# Autodesk Inventor assembly: TimingPulley_S5M_Mechalock
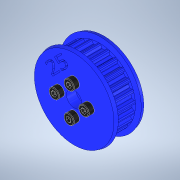
[picture p0: Inventor's stored thumbnail of the model, 180x180]
Saved by Autodesk Inventor 2022 (Build 260153000, 153)
## iProperties
Created: 2022-03-19
Part Number: TimingPulley_S5M_Mechalock
Document SubType Name: Assembly
Designer: satot
Author: satot
## Documents named in this file (6)
- C:\Users\satot\Documents\GrabCAD\NHK2022\BasicParts\TimingPullay\TimingPulley_S5M_Mechalock\TimingPulley_S5M_Mechalock.iam
- C:\Users\satot\Documents\GrabCAD\NHK2022\BasicParts\TimingPullay\TimingPulley_S5M_Mechalock\TimingPulley_S5M_MechaLock_2.ipt
- C:\Users\satot\Documents\GrabCAD\NHK2022\Content Center Files\R2022\ja-JP\六角穴付きボルト\六角穴付きボルト - M3 × 20 - 0.5.ipt
- C:\Users\satot\Documents\GrabCAD\NHK2022\Content Center Files\R2022\ja-JP\スプリング\スプリング - M3 × 0.7.ipt
- C:\Users\satot\Documents\GrabCAD\NHK2022\Content Center Files\R2022\ja-JP\ナット\ナット - M3 × 2.4.ipt
- C:\Users\satot\Documents\GrabCAD\NHK2022\BasicParts\TimingPullay\TimingPulley_S5M_Mechalock\TimingPulley_S5M_MechaLock_1.ipt
## Components (14 placed, 5 different names)
1. TimingPulley_S5M_MechaLock_1:1 — フラッシュ:1, メイト:1, メイト:2, メイト:3, メイト:4, メイト:5, メイト:6, メイト:7, メイト:8, メイト:9, メイト:10, メイト:11, メイト:13, メイト:15, メイト:17
2. TimingPulley_S5M_MechaLock_2:1 — フラッシュ:1, メイト:1, メイト:2, メイト:12, メイト:14, メイト:16, メイト:18
3. 六角穴付きボルト M3 x 20:1 — メイト:3, メイト:4
4. スプリング M3:1 — メイト:11, メイト:12, 挿入:1
5. ナット M3:1 — 挿入:1
6. 六角穴付きボルト M3 x 20:2 — メイト:5, メイト:6
7. 六角穴付きボルト M3 x 20:3 — メイト:7, メイト:8
8. 六角穴付きボルト M3 x 20:4 — メイト:9, メイト:10
9. スプリング M3:2 — メイト:13, メイト:14, 挿入:2
10. スプリング M3:3 — メイト:15, メイト:16, 挿入:3
11. スプリング M3:4 — メイト:17, メイト:18, 挿入:4
12. ナット M3:2 — 挿入:2
13. ナット M3:3 — 挿入:3
14. ナット M3:4 — 挿入:4
## Relationships (23: Mate 18, Insert 4, Flush 1)
- フラッシュ:1 [Flush] (-1.143 mm): TimingPulley_S5M_MechaLock_1:1 ↔ TimingPulley_S5M_MechaLock_2:1
- メイト:1 [Mate]: TimingPulley_S5M_MechaLock_1:1 ↔ TimingPulley_S5M_MechaLock_2:1
- メイト:2 [Mate]: TimingPulley_S5M_MechaLock_1:1 ↔ TimingPulley_S5M_MechaLock_2:1
- メイト:3 [Mate]: TimingPulley_S5M_MechaLock_1:1 ↔ 六角穴付きボルト M3 x 20:1
- メイト:4 [Mate]: TimingPulley_S5M_MechaLock_1:1 ↔ 六角穴付きボルト M3 x 20:1
- メイト:5 [Mate]: TimingPulley_S5M_MechaLock_1:1 ↔ 六角穴付きボルト M3 x 20:2
- メイト:6 [Mate]: TimingPulley_S5M_MechaLock_1:1 ↔ 六角穴付きボルト M3 x 20:2
- メイト:7 [Mate]: TimingPulley_S5M_MechaLock_1:1 ↔ 六角穴付きボルト M3 x 20:3
- メイト:8 [Mate]: TimingPulley_S5M_MechaLock_1:1 ↔ 六角穴付きボルト M3 x 20:3
- メイト:9 [Mate]: TimingPulley_S5M_MechaLock_1:1 ↔ 六角穴付きボルト M3 x 20:4
- メイト:10 [Mate]: TimingPulley_S5M_MechaLock_1:1 ↔ 六角穴付きボルト M3 x 20:4
- メイト:11 [Mate]: TimingPulley_S5M_MechaLock_1:1 ↔ スプリング M3:1
- メイト:12 [Mate]: TimingPulley_S5M_MechaLock_2:1 ↔ スプリング M3:1
- メイト:13 [Mate]: TimingPulley_S5M_MechaLock_1:1 ↔ スプリング M3:2
- メイト:14 [Mate]: TimingPulley_S5M_MechaLock_2:1 ↔ スプリング M3:2
- メイト:15 [Mate]: TimingPulley_S5M_MechaLock_1:1 ↔ スプリング M3:3
- メイト:16 [Mate]: TimingPulley_S5M_MechaLock_2:1 ↔ スプリング M3:3
- メイト:17 [Mate]: TimingPulley_S5M_MechaLock_1:1 ↔ スプリング M3:4
- メイト:18 [Mate]: TimingPulley_S5M_MechaLock_2:1 ↔ スプリング M3:4
- 挿入:1 [Insert]: スプリング M3:1 ↔ ナット M3:1
- 挿入:2 [Insert]: スプリング M3:2 ↔ ナット M3:2
- 挿入:3 [Insert]: スプリング M3:3 ↔ ナット M3:3
- 挿入:4 [Insert]: スプリング M3:4 ↔ ナット M3:4
